# Autodesk Inventor assembly: Extruder_Asem
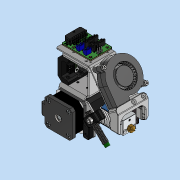
[picture p0: Inventor's stored thumbnail of the model, 180x180]
Saved by Autodesk Inventor 2020 (Build 240168000, 168)
## iProperties
Created: 2021-05-03
Part Number: Extruder_Asem
Document SubType Name: Assembly
Designer: ken113
Author: ken113
## Documents named in this file (16)
- C:\Users\lvglv\Documents\GitHub\Cheap_Belt_Printer\Model\Asem\Extruder_Asem.iam
- C:\Users\lvglv\Documents\GitHub\Cheap_Belt_Printer\Model\Parts\Meviy\Gantry_Angle.ipt
- C:\Users\lvglv\Documents\GitHub\Cheap_Belt_Printer\Model\Parts\Extruder\artillery-sidewinder-x1-v4-bondtech-bmg-with-e3d-lite-6-fan-holder-and-duct-1.snapshot.5\Bondtech BMG v5.iam
- C:\Users\lvglv\Documents\GitHub\Cheap_Belt_Printer\Model\Parts\Stepper Motor\NEMA17\Nema 17HS4401-S.ipt
- C:\Users\lvglv\Documents\GitHub\Cheap_Belt_Printer\Model\Parts\Electrical_Components\Radial Cooling Fan 50mm DC12V\Radial-Cooling-Fan-5015-DC12V.iam
- C:\Users\lvglv\Documents\GitHub\Cheap_Belt_Printer\Model\Parts\Hotend\Mixing_Hotend\Mixing_Hotend.iam
- C:\Users\lvglv\Documents\GitHub\Cheap_Belt_Printer\Model\Parts\Electrical_Components\inductive-sensor-m8-1.snapshot.4\Sensor Indutivo M8.iam
- C:\Users\lvglv\Documents\GitHub\Cheap_Belt_Printer\Model\Parts\Print_Parts\Rev3_Parts\Sensor_Holder.ipt
- C:\Users\lvglv\Documents\GitHub\Cheap_Belt_Printer\Model\Parts\Electrical_Components\lerdge-micro-switch-1.snapshot.2\endstop.ipt
- C:\Users\lvglv\Documents\GitHub\Cheap_Belt_Printer\Model\Parts\Print_Parts\Rev3_Parts\X_End_Holder.ipt
- C:\Users\lvglv\Documents\GitHub\Cheap_Belt_Printer\Model\Parts\Bolt\M3 x 18.ipt
- C:\Users\lvglv\Documents\GitHub\Cheap_Belt_Printer\Model\Parts\Bolt\M4 x 10.ipt
- C:\Users\lvglv\Documents\GitHub\Cheap_Belt_Printer\Model\Parts\Meviy\Fan_Holder.ipt
- C:\Users\lvglv\Documents\GitHub\Cheap_Belt_Printer\Model\Parts\PCB\Hotend_PCB\Hotend_PCB.iam
- C:\Users\lvglv\Documents\GitHub\Cheap_Belt_Printer\Model\Parts\Hotend\E3D_V6\e3d-v6-1-75mm-hotend-assembly-mockup-1.snapshot.4\Fan Assembly.iam
- C:\Users\lvglv\Documents\GitHub\Cheap_Belt_Printer\Model\Parts\Print_Parts\Rev3_Parts\Fan_Holder_A.ipt
## Components (16 placed, 15 different names)
1. Gantry_Angle:1 — 挿入:3, メイト:2, 角度:2, 挿入:5, 挿入:6, 角度:4, 角度:5, 挿入:10, 挿入:11, メイト:5, フラッシュ:3, 角度:7, 角度:8, メイト:8
2. Bondtech BMG v5:1 [sub-assembly] — 挿入:4, 角度:6
3. Nema 17HS4401-S:1 — 挿入:3, メイト:2
4. Mixing_Hotend:1 [sub-assembly] — 挿入:4, 角度:4, 挿入:19
5. Radial-Cooling-Fan-5015-DC12V:1 [sub-assembly] — 角度:2, 挿入:13, 挿入:14, 挿入:20
6. Sensor Indutivo M8:1 [sub-assembly] — メイト:3, フラッシュ:1
7. Sensor_Holder:1 — 挿入:5, 挿入:6, メイト:3, フラッシュ:1, 挿入:15
8. endstop:1 — 角度:5, 挿入:12
9. X_End_Holder:1 — 挿入:10, 挿入:11, 挿入:12
10. AS 1420 - Metric M3 x 18:1 — 挿入:13
11. AS 1420 - Metric M3 x 18:2 — 挿入:14
12. AS 1420 - Metric M4 x 10:1 — 挿入:15
13. Fan_Holder:3 — メイト:5, フラッシュ:3, 挿入:20, 挿入:21, 挿入:22, メイト:6, メイト:7, メイト:8
14. Fan Assembly:1 [sub-assembly] — 挿入:19, 角度:6
15. Hotend_PCB:1 [sub-assembly] — 角度:7, 角度:8, メイト:6, メイト:7
16. Fan_Holder_A:1 — 挿入:21, 挿入:22
## Relationships (30: Insert 15, Mate 7, Angle 6, Flush 2)
- [Mate]: Bondtech BMG v5:1 ↔ Nema 17HS4401-S:1
- [Insert] (2 mm): Bondtech BMG v5:1 ↔ Nema 17HS4401-S:1
- 挿入:3 [Insert]: Gantry_Angle:1 ↔ Nema 17HS4401-S:1
- メイト:2 [Mate]: Gantry_Angle:1 ↔ Nema 17HS4401-S:1
- 挿入:4 [Insert]: Bondtech BMG v5:1 ↔ Mixing_Hotend:1
- 角度:2 [Angle] (0 deg): Gantry_Angle:1 ↔ Radial-Cooling-Fan-5015-DC12V:1
- 挿入:5 [Insert]: Gantry_Angle:1 ↔ Sensor_Holder:1
- 挿入:6 [Insert]: Gantry_Angle:1 ↔ Sensor_Holder:1
- 角度:4 [Angle] (0 deg): Gantry_Angle:1 ↔ Mixing_Hotend:1
- メイト:3 [Mate]: Sensor Indutivo M8:1 ↔ Sensor_Holder:1
- フラッシュ:1 [Flush] (4 mm): Sensor Indutivo M8:1 ↔ Sensor_Holder:1
- 角度:5 [Angle] (180 deg): Gantry_Angle:1 ↔ endstop:1
- 挿入:10 [Insert]: Gantry_Angle:1 ↔ X_End_Holder:1
- 挿入:11 [Insert]: Gantry_Angle:1 ↔ X_End_Holder:1
- 挿入:12 [Insert]: endstop:1 ↔ X_End_Holder:1
- 挿入:13 [Insert]: Radial-Cooling-Fan-5015-DC12V:1 ↔ AS 1420 - Metric M3 x 18:1
- 挿入:14 [Insert]: Radial-Cooling-Fan-5015-DC12V:1 ↔ AS 1420 - Metric M3 x 18:2
- 挿入:15 [Insert]: Sensor_Holder:1 ↔ AS 1420 - Metric M4 x 10:1
- メイト:5 [Mate] (3 mm): Gantry_Angle:1 ↔ Fan_Holder:3
- フラッシュ:3 [Flush]: Gantry_Angle:1 ↔ Fan_Holder:3
- 挿入:19 [Insert]: Mixing_Hotend:1 ↔ Fan Assembly:1
- 角度:6 [Angle] (0 deg): Bondtech BMG v5:1 ↔ Fan Assembly:1
- 角度:7 [Angle] (180 deg): Gantry_Angle:1 ↔ Hotend_PCB:1
- 角度:8 [Angle] (180 deg): Gantry_Angle:1 ↔ Hotend_PCB:1
- 挿入:20 [Insert]: Radial-Cooling-Fan-5015-DC12V:1 ↔ Fan_Holder:3
- 挿入:21 [Insert]: Fan_Holder:3 ↔ Fan_Holder_A:1
- 挿入:22 [Insert]: Fan_Holder:3 ↔ Fan_Holder_A:1
- メイト:6 [Mate] (5 mm): Fan_Holder:3 ↔ Hotend_PCB:1
- メイト:7 [Mate]: Fan_Holder:3 ↔ Hotend_PCB:1
- メイト:8 [Mate]: Gantry_Angle:1 ↔ Fan_Holder:3
## Named parameters: d513_d217_d166 = 0 mm, d514_d218_d167 = 2 mm
